# Autodesk Inventor assembly: Сборка
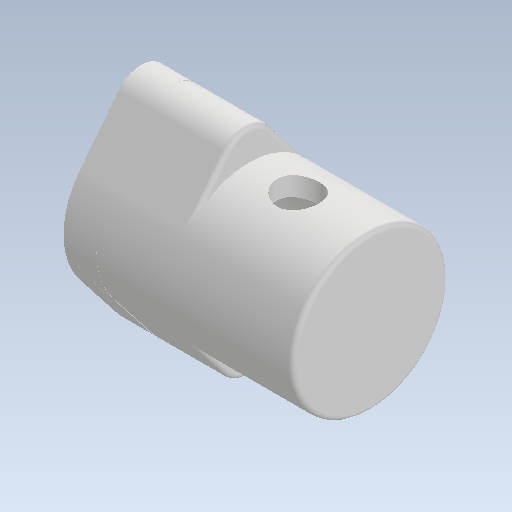
[picture p0: Inventor's stored thumbnail of the model, 512x512]
Saved by Autodesk Inventor 2021 (Build 250183000, 183)
## iProperties
Created: 2021-03-24
Part Number: Сборка
Document SubType Name: Assembly
Designer: khosta
Mass: 244.841 g
Surface Area: 549.512 cm^2
Volume: 208.922 cm^3
Density: 1.17192 g/cm^3
Author: khosta
## Documents named in this file (4)
- D:\Институт\Инженерная графика\Сборка 13В\Sborka.iam
- D:\Институт\Инженерная графика\Сборка 13В\Sborka_13V_kastryulya.ipt
- D:\Институт\Инженерная графика\Сборка 13В\Sborka_13V_kryshka.ipt
- C:\Users\khost\Documents\Inventor\Content Center Files\R2021\ru-RU\GOST 1491-80 B\Винт M10x1,25-6gx20 ГОСТ 1491-80.ipt
## Components (4 placed, 3 different names)
1. Sborka_13V_kastryulya:1 — С поворотом:1
2. Sborka_13V_kryshka:1 — С поворотом:1, Вставка:1, Вставка:2
3. Винт 2 ГОСТ 1491-80 M10 x 1,25 x 20:1 — Вставка:1
4. Винт 2 ГОСТ 1491-80 M10 x 1,25 x 20:2 — Вставка:2
## Relationships (3: Insert 2, RevoluteJoint 1)
- С поворотом:1 [RevoluteJoint]: Sborka_13V_kastryulya:1 ↔ Sborka_13V_kryshka:1
- Вставка:1 [Insert]: Sborka_13V_kryshka:1 ↔ Винт 2 ГОСТ 1491-80 M10 x 1,25 x 20:1
- Вставка:2 [Insert]: Sborka_13V_kryshka:1 ↔ Винт 2 ГОСТ 1491-80 M10 x 1,25 x 20:2
